# Autodesk Inventor assembly: Montagem do Motor Radial
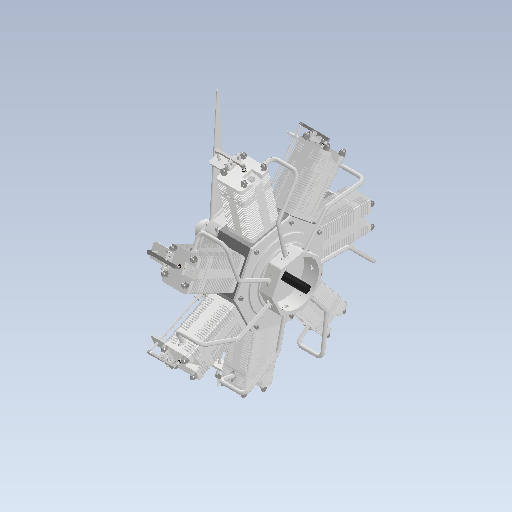
[picture p0: Inventor's stored thumbnail of the model, 512x512]
Saved by Autodesk Inventor 2021 (Build 250183000, 183)
## iProperties
Category: 1
Created: 2021-07-26
Document SubType Name: Assembly
Designer: Giovanni
Checked By: Prof. Luis
User Status: 1:15
Author: Giovanni Rodrigues Dias
Title: Montagem do Motor Radial
Keywords: 1
## Documents named in this file (34)
- C:\Users\irineu\Documents\Inventor\MotorRadial7\MontagemFinal2.iam
- C:\Users\irineu\Documents\Inventor\MotorRadial7\Peça4.ipt
- C:\Users\irineu\Documents\Inventor\Content Center Files\R2021\pt-BR\DIN BEARING(1)\DIN 625 SKF - SKF 6008.ipt
- C:\Users\irineu\Documents\Inventor\MotorRadial7\Conjunto_Virabrequim.iam
- C:\Users\irineu\Documents\Inventor\MotorRadial7\BielaMestraEquipada.iam
- C:\Users\irineu\Documents\Inventor\MotorRadial7\PistaoEquipado.iam
- C:\Users\irineu\Documents\Inventor\MotorRadial7\BielaArticuladaEquipada.iam
- C:\Users\irineu\Documents\Inventor\MotorRadial7\Pino de Ligação.ipt
- C:\Users\irineu\Documents\Inventor\MotorRadial7\Peça38.ipt
- C:\Users\irineu\Documents\Inventor\MotorRadial7\Peça6.ipt
- C:\Users\irineu\Documents\Inventor\MotorRadial7\Peça34.ipt
- C:\Users\irineu\Documents\Inventor\MotorRadial7\Superior do cilindro 2.iam
- C:\Users\irineu\Documents\Inventor\Content Center Files\R2021\pt-BR\DIN 1587\DIN 1587 - M16 x 2.ipt
- C:\Users\irineu\Documents\Inventor\MotorRadial7\Peça42.ipt
- C:\Users\irineu\Documents\Inventor\MotorRadial7\Peça20.3.ipt
- C:\Users\irineu\Documents\Inventor\Content Center Files\R2021\pt-BR\DIN 6885-1 A\DIN 6885 - A 12 x 8 x 32.ipt
- C:\Users\irineu\Documents\Inventor\MotorRadial7\Engrenagens.iam
- C:\Users\irineu\Documents\Inventor\MotorRadial7\Peça41.ipt
- C:\Users\irineu\Documents\Inventor\Content Center Files\R2021\pt-BR\DIN 912\DIN 912 - M4 x 0,7 x 10 x 8,25.ipt
- C:\Users\irineu\Documents\Inventor\MotorRadial7\Engrenagens 2.iam
- C:\Users\irineu\Documents\Inventor\MotorRadial7\Peça43.ipt
- C:\Users\irineu\Documents\Inventor\Content Center Files\R2021\pt-BR\DIN 471(2)\DIN 471 - 20 x 1,2(1).ipt
- C:\Users\irineu\Documents\Inventor\MotorRadial7\Peça44.ipt
- C:\Users\irineu\Documents\Inventor\MotorRadial7\Conjunto de Came.iam
- C:\Users\irineu\Documents\Inventor\Content Center Files\R2021\pt-BR\DIN 6885-1 A\DIN 6885 - A 12 x 8 x 45.ipt
- C:\Users\irineu\Documents\Inventor\MotorRadial7\Peça35.ipt
- C:\Users\irineu\Documents\Inventor\Content Center Files\R2021\pt-BR\DIN 471(2)\DIN 471 - 40 x 1,75(1).ipt
- C:\Users\irineu\Documents\Inventor\MotorRadial7\Peça36.ipt
- C:\Users\irineu\Documents\Inventor\MotorRadial7\Peça37.ipt
- C:\Users\irineu\Documents\Inventor\MotorRadial7\Conexão2.iam
- C:\Users\irineu\Documents\Inventor\MotorRadial7\Peça33.ipt
- C:\Users\irineu\Documents\Inventor\MotorRadial7\Tubo auxiliar 2.iam
- C:\Users\irineu\Documents\Inventor\Content Center Files\R2021\pt-BR\DIN 912\DIN 912 - M12 x 1,75 x 25 x 20,625.ipt
- C:\Users\irineu\Documents\Inventor\Content Center Files\R2021\pt-BR\DIN 912\DIN 912 - M8 x 1,25 x 20 x 16,875.ipt
## Components (184 placed, 33 different names)
1. Peça4:1 — Alinhado:1, Alinhado:2, Alinhado:3, Inserir:1, Coincidente:2, Coincidente:4, Coincidente:6, Coincidente:8, Coincidente:10, Coincidente:12, Coincidente:14, Inserir:16, Inserir:17, Ângulo:2, Inserir:22, Ângulo:5, Inserir:46, Alinhado:6
2. DIN 625 SKF SKF 6008:1 — Inserir:1, Inserir:2, Inserir:21
3. Conjunto_Virabrequim:1 [sub-assembly] — Inserir:2, Inserir:3, Ângulo:1, Inserir:23, Coincidente:15, Inserir:33, Coincidente:22, Inserir:35, Inserir:36, Coincidente:24, Alinhado:5, Inserir:45
4. BielaMestraEquipada:1 [sub-assembly] — Inserir:3, Coincidente:1, Inserir:4, Inserir:5, Inserir:6, Inserir:7, Inserir:8, Inserir:9, Inserir:10, Inserir:11, Inserir:12, Inserir:13, Inserir:14, Inserir:15
5. PistaoEquipado:1 [sub-assembly] — Coincidente:1, Coincidente:2
6. PistaoEquipado:2 [sub-assembly] — Coincidente:3, Coincidente:4
7. PistaoEquipado:3 [sub-assembly] — Coincidente:5, Coincidente:6
8. PistaoEquipado:4 [sub-assembly] — Coincidente:7, Coincidente:8
9. PistaoEquipado:5 [sub-assembly] — Coincidente:9, Coincidente:10
10. PistaoEquipado:6 [sub-assembly] — Coincidente:11, Coincidente:12
11. PistaoEquipado:7 [sub-assembly] — Coincidente:13, Coincidente:14
12. BielaArticuladaEquipada:1 [sub-assembly] — Inserir:4, Coincidente:3
13. BielaArticuladaEquipada:2 [sub-assembly] — Inserir:6, Coincidente:5
14. BielaArticuladaEquipada:3 [sub-assembly] — Inserir:7, Coincidente:7
15. BielaArticuladaEquipada:4 [sub-assembly] — Inserir:8, Coincidente:9
16. BielaArticuladaEquipada:5 [sub-assembly] — Inserir:9, Coincidente:11
17. BielaArticuladaEquipada:6 [sub-assembly] — Inserir:10, Coincidente:13
18. Pino_de_Ligação1:1 — Inserir:5
19. Pino_de_Ligação1:2 — Inserir:12
20. Pino_de_Ligação1:3 — Inserir:13
21. Pino_de_Ligação1:4 — Inserir:14
22. Pino_de_Ligação1:5 — Inserir:11
23. Pino_de_Ligação1:6 — Inserir:15
24. Peça42:1 — Inserir:21, Inserir:24
25. Peça20.3:1 — Inserir:22, Ângulo:5, Inserir:25, Coincidente:17, Coincidente:18, Inserir:34, Coincidente:23, Inserir:38, Inserir:39, Inserir:40, Inserir:41, Inserir:42, Inserir:43, Inserir:44, Inserir:57
26. DIN 6885-1 A A 12 x 8 x 32:1 — Inserir:23, Coincidente:15
27. Engrenagens:1 [sub-assembly] — Inserir:24, Rotação:1, Coincidente:19, Inserir:30
28. Peça41:1 — Inserir:25, Coincidente:17, Coincidente:18, Inserir:26, Inserir:27, Inserir:29
29. Engrenagens 2:1 [sub-assembly] — Inserir:27, Rotação:1, Coincidente:19, Inserir:28, Coincidente:20, Coincidente:21, Rotação:2
30. Peça43:1 — Inserir:28
31. DIN 471 > 9mm <= 300mm 20 x 1,2:1 — Inserir:29, Coincidente:20
32. Peça44:1 — Inserir:30, Inserir:31
33. Conjunto de Came:1 [sub-assembly] — Inserir:31, Coincidente:21, Rotação:2
34. DIN 6885-1 A A 12 x 8 x 45:1 — Inserir:33, Coincidente:22
35. Peça35:1 — Inserir:34, Coincidente:23, Inserir:58
36. DIN 471 > 9mm <= 300mm 40 x 1,75:1 — Inserir:35
37. Peça36:1 — Inserir:36, Coincidente:24, Inserir:37
38. Peça37:1 — Inserir:37, Alinhado:5
39. Conexão2:1 [sub-assembly] — Inserir:38, Ângulo:6
40. Conexão2:2 [sub-assembly] — Inserir:39, Ângulo:7
41. Conexão2:3 [sub-assembly] — Inserir:40, Ângulo:8
42. Conexão2:4 [sub-assembly] — Inserir:41, Ângulo:9
43. Conexão2:5 [sub-assembly] — Inserir:42, Ângulo:10
44. Conexão2:6 [sub-assembly] — Inserir:43, Ângulo:11
45. Conexão2:7 [sub-assembly] — Inserir:44, Ângulo:12
46. DIN 625 SKF SKF 6008:2 — Inserir:45
47. Peça33:1 — Inserir:46, Alinhado:6, Inserir:56
48. Peça6:1 — Inserir:17, Ângulo:2, Inserir:18, Alinhado:4, Ângulo:4
49. Peça34:1 — Inserir:18, Alinhado:4, Inserir:19
50. Superior do cilindro 2:1 [sub-assembly] — Inserir:19, Inserir:20, Ângulo:3, Ângulo:4, Ângulo:11
51. Peça6:2
52. Peça34:2
53. Superior do cilindro 2:2 [sub-assembly] — Ângulo:12
54. Peça6:3
55. Peça34:3
56. Superior do cilindro 2:3 [sub-assembly] — Ângulo:6, Inserir:59, Coincidente:25
57. Peça6:4
58. Peça34:4
59. Superior do cilindro 2:4 [sub-assembly] — Ângulo:7
60. Peça6:5
61. Peça34:5
62. Superior do cilindro 2:5 [sub-assembly] — Ângulo:8
63. Peça6:6
64. Peça34:6
65. Superior do cilindro 2:6 [sub-assembly] — Ângulo:9
66. Peça6:7
67. Peça34:7
68. Superior do cilindro 2:7 [sub-assembly] — Ângulo:10
69. DIN 912 - substituído por DIN EN ISO 4762 M4 x 10:1 — Inserir:26
70. DIN 912 - substituído por DIN EN ISO 4762 M4 x 10:2
71. DIN 912 - substituído por DIN EN ISO 4762 M4 x 10:3
72. DIN 912 - substituído por DIN EN ISO 4762 M4 x 10:4
73. DIN 912 - substituído por DIN EN ISO 4762 M12 x 25:1 — Inserir:56
74. DIN 912 - substituído por DIN EN ISO 4762 M12 x 25:2 — Inserir:57
75. DIN 912 - substituído por DIN EN ISO 4762 M12 x 25:3
76. DIN 912 - substituído por DIN EN ISO 4762 M12 x 25:4
77. DIN 912 - substituído por DIN EN ISO 4762 M12 x 25:5
78. DIN 912 - substituído por DIN EN ISO 4762 M12 x 25:6
79. DIN 912 - substituído por DIN EN ISO 4762 M12 x 25:7
80. DIN 912 - substituído por DIN EN ISO 4762 M12 x 25:8
81. DIN 912 - substituído por DIN EN ISO 4762 M12 x 25:9
82. DIN 912 - substituído por DIN EN ISO 4762 M12 x 25:10
83. DIN 912 - substituído por DIN EN ISO 4762 M12 x 25:11
84. DIN 912 - substituído por DIN EN ISO 4762 M12 x 25:12
85. DIN 912 - substituído por DIN EN ISO 4762 M12 x 25:13
86. DIN 912 - substituído por DIN EN ISO 4762 M12 x 25:14
87. DIN 912 - substituído por DIN EN ISO 4762 M8 x 20:1 — Inserir:58
88. DIN 912 - substituído por DIN EN ISO 4762 M8 x 20:2
89. DIN 912 - substituído por DIN EN ISO 4762 M8 x 20:3
90. DIN 912 - substituído por DIN EN ISO 4762 M8 x 20:4
91. DIN 912 - substituído por DIN EN ISO 4762 M8 x 20:5
92. DIN 912 - substituído por DIN EN ISO 4762 M8 x 20:6
93. DIN 912 - substituído por DIN EN ISO 4762 M8 x 20:7
94. Tubo auxiliar 2:1 [sub-assembly] — Inserir:59, Coincidente:25, Inserir:60, Inserir:61, Inserir:62, Inserir:63
95. DIN 912 - substituído por DIN EN ISO 4762 M4 x 10:11 — Inserir:63
96. DIN 912 - substituído por DIN EN ISO 4762 M4 x 10:12 — Inserir:62
97. DIN 912 - substituído por DIN EN ISO 4762 M4 x 10:13 — Inserir:61
98. DIN 912 - substituído por DIN EN ISO 4762 M4 x 10:14 — Inserir:60
99. Tubo auxiliar 2:2 [sub-assembly]
100. DIN 912 - substituído por DIN EN ISO 4762 M4 x 10:15
101. DIN 912 - substituído por DIN EN ISO 4762 M4 x 10:16
102. DIN 912 - substituído por DIN EN ISO 4762 M4 x 10:17
103. DIN 912 - substituído por DIN EN ISO 4762 M4 x 10:18
104. Tubo auxiliar 2:3 [sub-assembly]
105. DIN 912 - substituído por DIN EN ISO 4762 M4 x 10:19
106. DIN 912 - substituído por DIN EN ISO 4762 M4 x 10:20
107. DIN 912 - substituído por DIN EN ISO 4762 M4 x 10:21
108. DIN 912 - substituído por DIN EN ISO 4762 M4 x 10:22
109. Tubo auxiliar 2:4 [sub-assembly]
110. DIN 912 - substituído por DIN EN ISO 4762 M4 x 10:23
111. DIN 912 - substituído por DIN EN ISO 4762 M4 x 10:24
112. DIN 912 - substituído por DIN EN ISO 4762 M4 x 10:25
113. DIN 912 - substituído por DIN EN ISO 4762 M4 x 10:26
114. Tubo auxiliar 2:5 [sub-assembly]
115. DIN 912 - substituído por DIN EN ISO 4762 M4 x 10:27
116. DIN 912 - substituído por DIN EN ISO 4762 M4 x 10:28
117. DIN 912 - substituído por DIN EN ISO 4762 M4 x 10:29
118. DIN 912 - substituído por DIN EN ISO 4762 M4 x 10:30
119. Tubo auxiliar 2:6 [sub-assembly]
120. DIN 912 - substituído por DIN EN ISO 4762 M4 x 10:31
121. DIN 912 - substituído por DIN EN ISO 4762 M4 x 10:32
122. DIN 912 - substituído por DIN EN ISO 4762 M4 x 10:33
123. DIN 912 - substituído por DIN EN ISO 4762 M4 x 10:34
124. Tubo auxiliar 2:7 [sub-assembly]
125. DIN 912 - substituído por DIN EN ISO 4762 M4 x 10:35
126. DIN 912 - substituído por DIN EN ISO 4762 M4 x 10:36
127. DIN 912 - substituído por DIN EN ISO 4762 M4 x 10:37
128. DIN 912 - substituído por DIN EN ISO 4762 M4 x 10:38
129. Peça38:1 — Inserir:16
130. DIN 1587 M16:1 — Inserir:20, Ângulo:3
131. Peça38:2
132. DIN 1587 M16:2
133. Peça38:3
134. DIN 1587 M16:3
135. Peça38:4
136. DIN 1587 M16:4
137. Peça38:5
138. DIN 1587 M16:5
139. Peça38:6
140. DIN 1587 M16:6
141. Peça38:7
142. DIN 1587 M16:7
143. Peça38:8
144. DIN 1587 M16:8
145. Peça38:9
146. DIN 1587 M16:9
147. Peça38:10
148. DIN 1587 M16:10
149. Peça38:11
150. DIN 1587 M16:11
151. Peça38:12
152. DIN 1587 M16:12
153. Peça38:13
154. DIN 1587 M16:13
155. Peça38:14
156. DIN 1587 M16:14
157. Peça38:15
158. DIN 1587 M16:15
159. Peça38:16
160. DIN 1587 M16:16
161. Peça38:17
162. DIN 1587 M16:17
163. Peça38:18
164. DIN 1587 M16:18
165. Peça38:19
166. DIN 1587 M16:19
167. Peça38:20
168. DIN 1587 M16:20
169. Peça38:21
170. DIN 1587 M16:21
171. Peça38:22
172. DIN 1587 M16:22
173. Peça38:23
174. DIN 1587 M16:23
175. Peça38:24
176. DIN 1587 M16:24
177. Peça38:25
178. DIN 1587 M16:25
179. Peça38:26
180. DIN 1587 M16:26
181. Peça38:27
182. DIN 1587 M16:27
183. Peça38:28
184. DIN 1587 M16:28
## Component patterns: (7 elements, first: Peça6:1 + Peça34:1 + Superior do cilindro 2:1), (4 elements, first: DIN 912 - substituído por DIN EN ISO 4762 M4 x 10:1), (7 elements, first: DIN 912 - substituído por DIN EN ISO 4762 M12 x 25:1 + DIN 912 - substituído por DIN EN ISO 4762 M12 x 25:2), (7 elements, first: DIN 912 - substituído por DIN EN ISO 4762 M8 x 20:1), (7 elements, first: Tubo auxiliar 2:1 + DIN 912 - substituído por DIN EN ISO 4762 M4 x 10:11 + DIN 912 - substituído por DIN EN ISO 4762 M4 x 10:12 + DIN 912 - substituído por DIN EN ISO 4762 M4 x 10:13 + DIN 912 - substituído por DIN EN ISO 4762 M4 x 10:14), (4 elements, first: Peça38:1 + DIN 1587 M16:1), Componente de padrão 1:2 (4 elements), Componente de padrão 1:3 (4 elements), Componente de padrão 1:4 (4 elements), Componente de padrão 1:5 (4 elements), Componente de padrão 1:6 (4 elements), Componente de padrão 1:7 (4 elements)
## Relationships (97: Insert 53, Mate 24, Angle 12, Flush 6, RelateRotation 2)
- Alinhado:1 [Flush]: Peça4:1
- Alinhado:2 [Flush]: Peça4:1
- Alinhado:3 [Flush]: Peça4:1
- Inserir:1: Peça4:1 ↔ DIN 625 SKF SKF 6008:1
- Inserir:2: DIN 625 SKF SKF 6008:1 ↔ Conjunto_Virabrequim:1
- Inserir:3: Conjunto_Virabrequim:1 ↔ BielaMestraEquipada:1
- Coincidente:1 [Mate]: BielaMestraEquipada:1 ↔ PistaoEquipado:1
- Coincidente:2 [Mate]: Peça4:1 ↔ PistaoEquipado:1
- Inserir:4: BielaMestraEquipada:1 ↔ BielaArticuladaEquipada:1
- Coincidente:3 [Mate]: PistaoEquipado:2 ↔ BielaArticuladaEquipada:1
- Coincidente:4 [Mate]: Peça4:1 ↔ PistaoEquipado:2
- Inserir:5: BielaMestraEquipada:1 ↔ Pino_de_Ligação1:1
- Inserir:6: BielaMestraEquipada:1 ↔ BielaArticuladaEquipada:2
- Inserir:7: BielaMestraEquipada:1 ↔ BielaArticuladaEquipada:3
- Inserir:8: BielaMestraEquipada:1 ↔ BielaArticuladaEquipada:4
- Ângulo:1 [Angle] (0 deg): Conjunto_Virabrequim:1
- Inserir:9: BielaMestraEquipada:1 ↔ BielaArticuladaEquipada:5
- Inserir:10: BielaMestraEquipada:1 ↔ BielaArticuladaEquipada:6
- Inserir:11: BielaMestraEquipada:1 ↔ Pino_de_Ligação1:5
- Inserir:12: BielaMestraEquipada:1 ↔ Pino_de_Ligação1:2
- Inserir:13: BielaMestraEquipada:1 ↔ Pino_de_Ligação1:3
- Inserir:14: BielaMestraEquipada:1 ↔ Pino_de_Ligação1:4
- Inserir:15: BielaMestraEquipada:1 ↔ Pino_de_Ligação1:6
- Coincidente:5 [Mate]: PistaoEquipado:3 ↔ BielaArticuladaEquipada:2
- Coincidente:6 [Mate]: Peça4:1 ↔ PistaoEquipado:3
- Coincidente:7 [Mate]: PistaoEquipado:4 ↔ BielaArticuladaEquipada:3
- Coincidente:8 [Mate]: Peça4:1 ↔ PistaoEquipado:4
- Coincidente:9 [Mate]: PistaoEquipado:5 ↔ BielaArticuladaEquipada:4
- Coincidente:10 [Mate]: Peça4:1 ↔ PistaoEquipado:5
- Coincidente:11 [Mate]: PistaoEquipado:6 ↔ BielaArticuladaEquipada:5
- Coincidente:12 [Mate]: Peça4:1 ↔ PistaoEquipado:6
- Coincidente:13 [Mate]: PistaoEquipado:7 ↔ BielaArticuladaEquipada:6
- Coincidente:14 [Mate]: Peça4:1 ↔ PistaoEquipado:7
- Inserir:16: Peça4:1 ↔ Peça38:1
- Inserir:17: Peça4:1 ↔ Peça6:1
- Ângulo:2 [Angle] (0 deg): Peça4:1 ↔ Peça6:1
- Inserir:18: Peça6:1 ↔ Peça34:1
- Alinhado:4 [Flush]: Peça6:1 ↔ Peça34:1
- Inserir:19: Peça34:1 ↔ Superior do cilindro 2:1
- Inserir:20: Superior do cilindro 2:1 ↔ DIN 1587 M16:1
- Ângulo:3 [Angle] (0 deg): Superior do cilindro 2:1 ↔ DIN 1587 M16:1
- Ângulo:4 [Angle] (0 deg): Peça6:1 ↔ Superior do cilindro 2:1
- Inserir:21: DIN 625 SKF SKF 6008:1 ↔ Peça42:1
- Inserir:22: Peça4:1 ↔ Peça20.3:1
- Ângulo:5 [Angle] (0 deg): Peça4:1 ↔ Peça20.3:1
- Inserir:23: Conjunto_Virabrequim:1 ↔ DIN 6885-1 A A 12 x 8 x 32:1
- Coincidente:15 [Mate]: Conjunto_Virabrequim:1 ↔ DIN 6885-1 A A 12 x 8 x 32:1
- Inserir:24: Peça42:1 ↔ Engrenagens:1
- Inserir:25: Peça20.3:1 ↔ Peça41:1
- Coincidente:17 [Mate]: Peça20.3:1 ↔ Peça41:1
- Coincidente:18 [Mate]: Peça20.3:1 ↔ Peça41:1
- Inserir:26: Peça41:1 ↔ DIN 912 - substituído por DIN EN ISO 4762 M4 x 10:1
- Inserir:27: Peça41:1 ↔ Engrenagens 2:1
- Rotação:1 [RelateRotation] (1.56 ul): Engrenagens:1 ↔ Engrenagens 2:1
- Coincidente:19 [Mate]: Engrenagens:1 ↔ Engrenagens 2:1
- Inserir:28: Engrenagens 2:1 ↔ Peça43:1
- Inserir:29: Peça41:1 ↔ DIN 471 > 9mm <= 300mm 20 x 1,2:1
- Coincidente:20 [Mate]: Engrenagens 2:1 ↔ DIN 471 > 9mm <= 300mm 20 x 1,2:1
- Inserir:30: Engrenagens:1 ↔ Peça44:1
- Inserir:31: Peça44:1 ↔ Conjunto de Came:1
- Coincidente:21 [Mate]: Engrenagens 2:1 ↔ Conjunto de Came:1
- Rotação:2 [RelateRotation] (0.2809 ul): Engrenagens 2:1 ↔ Conjunto de Came:1
- Inserir:33: Conjunto_Virabrequim:1 ↔ DIN 6885-1 A A 12 x 8 x 45:1
- Coincidente:22 [Mate]: Conjunto_Virabrequim:1 ↔ DIN 6885-1 A A 12 x 8 x 45:1
- Inserir:34: Peça20.3:1 ↔ Peça35:1
- Coincidente:23 [Mate]: Peça20.3:1 ↔ Peça35:1
- Inserir:35: Conjunto_Virabrequim:1 ↔ DIN 471 > 9mm <= 300mm 40 x 1,75:1
- Inserir:36: Conjunto_Virabrequim:1 ↔ Peça36:1
- Coincidente:24 [Mate]: Conjunto_Virabrequim:1 ↔ Peça36:1
- Inserir:37: Peça36:1 ↔ Peça37:1
- Alinhado:5 [Flush]: Conjunto_Virabrequim:1 ↔ Peça37:1
- Inserir:38: Peça20.3:1 ↔ Conexão2:1
- Ângulo:6 [Angle] (180 deg): Conexão2:1 ↔ Superior do cilindro 2:3
- Inserir:39: Peça20.3:1 ↔ Conexão2:2
- Ângulo:7 [Angle] (180 deg): Conexão2:2 ↔ Superior do cilindro 2:4
- Inserir:40: Peça20.3:1 ↔ Conexão2:3
- Ângulo:8 [Angle] (180 deg): Conexão2:3 ↔ Superior do cilindro 2:5
- Inserir:41: Peça20.3:1 ↔ Conexão2:4
- Ângulo:9 [Angle] (180 deg): Conexão2:4 ↔ Superior do cilindro 2:6
- Inserir:42: Peça20.3:1 ↔ Conexão2:5
- Ângulo:10 [Angle] (180 deg): Conexão2:5 ↔ Superior do cilindro 2:7
- Inserir:43: Peça20.3:1 ↔ Conexão2:6
- Ângulo:11 [Angle] (180 deg): Conexão2:6 ↔ Superior do cilindro 2:1
- Inserir:44: Peça20.3:1 ↔ Conexão2:7
- Ângulo:12 [Angle] (180 deg): Conexão2:7 ↔ Superior do cilindro 2:2
- Inserir:45: Conjunto_Virabrequim:1 ↔ DIN 625 SKF SKF 6008:2
- Inserir:46: Peça4:1 ↔ Peça33:1
- Alinhado:6 [Flush]: Peça4:1 ↔ Peça33:1
- Inserir:56: Peça33:1 ↔ DIN 912 - substituído por DIN EN ISO 4762 M12 x 25:1
- Inserir:57: Peça20.3:1 ↔ DIN 912 - substituído por DIN EN ISO 4762 M12 x 25:2
- Inserir:58: Peça35:1 ↔ DIN 912 - substituído por DIN EN ISO 4762 M8 x 20:1
- Inserir:59: Superior do cilindro 2:3 ↔ Tubo auxiliar 2:1
- Coincidente:25 [Mate]: Superior do cilindro 2:3 ↔ Tubo auxiliar 2:1
- Inserir:60: Tubo auxiliar 2:1 ↔ DIN 912 - substituído por DIN EN ISO 4762 M4 x 10:14
- Inserir:61: Tubo auxiliar 2:1 ↔ DIN 912 - substituído por DIN EN ISO 4762 M4 x 10:13
- Inserir:62: Tubo auxiliar 2:1 ↔ DIN 912 - substituído por DIN EN ISO 4762 M4 x 10:12
- Inserir:63: Tubo auxiliar 2:1 ↔ DIN 912 - substituído por DIN EN ISO 4762 M4 x 10:11
